# Autodesk Inventor assembly: GripE
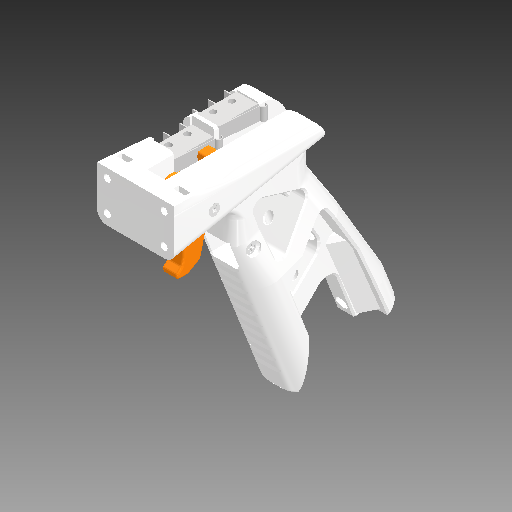
[picture p0: Inventor's stored thumbnail of the model, 512x512]
Saved by Autodesk Inventor 2020 (Build 240168000, 168)
## iProperties
Created: 2020-09-14
Part Number: GripE
Document SubType Name: Assembly
Designer: DDeGo
Author: DDeGo
Revision Number: PRODUCT_VERSION_IDPRODUCT_VERSION_DESCR
## Documents named in this file (5)
- C:\Users\DDeGo\Documents\Drew\Projects\Nerf_Aimbot\ESPER\GripE.iam
- C:\Users\DDeGo\Documents\Drew\Projects\Nerf_Aimbot\ESPER\GripE.ipt
- C:\Users\DDeGo\Documents\Drew\Projects\Nerf_Aimbot\ESPER\TriggerE.ipt
- C:\Users\DDeGo\Documents\Drew\Projects\Nerf_Aimbot\ESPER\90273A108.ipt
- C:\Users\DDeGo\Documents\Drew\Projects\Nerf_Aimbot\Cad\E5 - Micro Endstop Triggered.ipt
## Components (8 placed, 7 different names)
1. NAUO_ID9 — Mate:1, Mate:2, Mate:3, Mate:4, Mate:5, Mate:6, Mate:7, Mate:8
2. NAUO_ID29 — Mate:1, Mate:2
3. NAUO_ID69
4. NAUO_ID79
5. NAUO_ID99
6. NAUO_ID109
7. E5 - Micro Endstop Triggered:1 — Mate:3, Mate:7, Mate:8
8. E5 - Micro Endstop Triggered:2 — Mate:4, Mate:5, Mate:6
## Relationships (8: Mate 8)
- Mate:1: NAUO_ID9 ↔ NAUO_ID29
- Mate:2 (0.75 mm): NAUO_ID9 ↔ NAUO_ID29
- Mate:3: NAUO_ID9 ↔ E5 - Micro Endstop Triggered:1
- Mate:4: NAUO_ID9 ↔ E5 - Micro Endstop Triggered:2
- Mate:5: NAUO_ID9 ↔ E5 - Micro Endstop Triggered:2
- Mate:6: NAUO_ID9 ↔ E5 - Micro Endstop Triggered:2
- Mate:7: NAUO_ID9 ↔ E5 - Micro Endstop Triggered:1
- Mate:8: NAUO_ID9 ↔ E5 - Micro Endstop Triggered:1
